# Autodesk Inventor assembly: Dash-V1
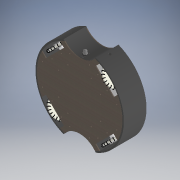
[picture p0: Inventor's stored thumbnail of the model, 180x180]
Saved by Autodesk Inventor 2020 (Build 240168000, 168)
## iProperties
Created: 2024-10-26
Part Number: Dash-V1
Document SubType Name: Assembly
Designer: Ivan
Mass: 1036.29 g
Surface Area: 3844.11 cm^2
Volume: 1024.75 cm^3
Density: 1.01126 g/cm^3
Author: Ivan
## Documents named in this file (13)
- C:\!projects\DASH_\3D\Dash-V1\Dash-V1.iam
- C:\!projects\DASH_\3D\Dash-V1\floor_v2.ipt
- C:\!projects\DASH_\3D\Dash-V1\motor_mount\motor_mount_edge_v2.ipt
- C:\!projects\DASH_\3D\Dash-V1\motor_mount\motor_converter.ipt
- C:\!projects\DASH_\3D\Dash-V1\motor_mount\motor_mount_part2_v2.ipt
- C:\!projects\DASH_\3D\Dash-V1\motor20.ipt
- C:\!projects\DASH_\3D\Dash-V1\wheel\Wheel.iam
- C:\!projects\DASH_\3D\Dash-V1\contour.ipt
- C:\!projects\DASH_\3D\Dash-V1\protect_v2.ipt
- C:\!projects\DASH_\3D\Dash-V1\ball.ipt
- C:\!projects\DASH_\3D\Dash-V1\catch_v2.ipt
- C:\!projects\DASH_\3D\Dash-V1\Solenoid\Solenoid.iam
- C:\!projects\DASH_\3D\Dash-V1\motherboard\motherboard_asm.iam
## Components (27 placed, 12 different names)
1. ball:1 — Касательность:1, Касательность:2
2. motherboard_asm:1 [sub-assembly] — Вставка:46, Вставка:47
3. floor_v2:1 — Совмещение:2, Вставка:1, Вставка:2, Совмещение:3, Угол:1, Вставка:3, Вставка:4, Вставка:10, Вставка:11, Вставка:12, Вставка:13, Вставка:14, Вставка:15, Вставка:16, Вставка:17, Вставка:18, Вставка:19, Вставка:20, Вставка:21, Касательность:1, Вставка:38, Вставка:39, Вставка:40, Вставка:41, Совмещение:4, Касательность:3, Касательность:4, Вставка:42, Вставка:43, Вставка:44, Вставка:45
4. contour:1 — Вставка:9, Касательность:2, Вставка:35, Вставка:46, Вставка:47
5. motor_converter:1 — Вставка:36, Вставка:37, Угол:3
6. motor_mount_edge_v2:2 — Вставка:18, Вставка:19, Вставка:24, Вставка:25, Вставка:28, Вставка:35
7. motor_mount_edge_v2:3 — Вставка:20, Вставка:21, Вставка:22, Вставка:23, Вставка:30
8. motor_mount_edge_v2:4 — Вставка:14, Вставка:15, Вставка:26, Вставка:27, Вставка:29
9. motor_mount_edge_v2:1 — Вставка:1, Вставка:2, Вставка:5, Вставка:6, Вставка:7, Вставка:9
10. motor_mount_part2_v2:5 — Вставка:16, Вставка:17
11. motor_mount_part2_v2:6 — Вставка:12, Вставка:13
12. motor_mount_part2_v2:7 — Вставка:10, Вставка:11, Вставка:37
13. motor_mount_part2_v2:4 — Вставка:3, Вставка:4, Вставка:36
14. motor20:2 — Вставка:22, Вставка:23
15. motor20:3 — Вставка:24, Вставка:25
16. motor20:4 — Вставка:26, Вставка:27
17. motor20:1 — Вставка:5, Вставка:6
18. Wheel:1 [sub-assembly] — Вставка:7
19. Wheel:2 [sub-assembly] — Вставка:30
20. Wheel:3 [sub-assembly] — Вставка:29
21. Wheel:4 [sub-assembly] — Вставка:28
22. catch_v2:2 — Вставка:40, Вставка:41
23. catch_v2:1 — Вставка:38, Вставка:39
24. protect_v2:2 — Вставка:44, Вставка:45
25. protect_v2:1 — Вставка:42, Вставка:43
26. Solenoid:2 [sub-assembly] — Угол:2, Заподлицо:1, Заподлицо:2, Касательность:4, Угол:3
27. Solenoid:1 [sub-assembly] — Угол:2, Заподлицо:1, Совмещение:4, Заподлицо:2, Касательность:3
## Relationships (54: Insert 42, Tangent 4, Mate 3, Angle 3, Flush 2)
- Совмещение:2 [Mate]: floor_v2:1
- Вставка:1 [Insert]: floor_v2:1 ↔ motor_mount_edge_v2:1
- Вставка:2 [Insert]: floor_v2:1 ↔ motor_mount_edge_v2:1
- Совмещение:3 [Mate]: floor_v2:1
- Угол:1 [Angle] (45 deg): floor_v2:1
- Вставка:3 [Insert]: floor_v2:1 ↔ motor_mount_part2_v2:4
- Вставка:4 [Insert]: floor_v2:1 ↔ motor_mount_part2_v2:4
- Вставка:5 [Insert]: motor_mount_edge_v2:1 ↔ motor20:1
- Вставка:6 [Insert]: motor_mount_edge_v2:1 ↔ motor20:1
- Вставка:7 [Insert]: motor_mount_edge_v2:1 ↔ Wheel:1
- Вставка:9 [Insert]: contour:1 ↔ motor_mount_edge_v2:1
- Вставка:10 [Insert]: floor_v2:1 ↔ motor_mount_part2_v2:7
- Вставка:11 [Insert]: floor_v2:1 ↔ motor_mount_part2_v2:7
- Вставка:12 [Insert]: floor_v2:1 ↔ motor_mount_part2_v2:6
- Вставка:13 [Insert]: floor_v2:1 ↔ motor_mount_part2_v2:6
- Вставка:14 [Insert]: floor_v2:1 ↔ motor_mount_edge_v2:4
- Вставка:15 [Insert]: floor_v2:1 ↔ motor_mount_edge_v2:4
- Вставка:16 [Insert]: floor_v2:1 ↔ motor_mount_part2_v2:5
- Вставка:17 [Insert]: floor_v2:1 ↔ motor_mount_part2_v2:5
- Вставка:18 [Insert]: floor_v2:1 ↔ motor_mount_edge_v2:2
- Вставка:19 [Insert]: floor_v2:1 ↔ motor_mount_edge_v2:2
- Вставка:20 [Insert]: floor_v2:1 ↔ motor_mount_edge_v2:3
- Вставка:21 [Insert]: floor_v2:1 ↔ motor_mount_edge_v2:3
- Вставка:22 [Insert]: motor_mount_edge_v2:3 ↔ motor20:2
- Вставка:23 [Insert]: motor_mount_edge_v2:3 ↔ motor20:2
- Вставка:24 [Insert]: motor_mount_edge_v2:2 ↔ motor20:3
- Вставка:25 [Insert]: motor_mount_edge_v2:2 ↔ motor20:3
- Вставка:26 [Insert]: motor_mount_edge_v2:4 ↔ motor20:4
- Вставка:27 [Insert]: motor_mount_edge_v2:4 ↔ motor20:4
- Вставка:28 [Insert]: motor_mount_edge_v2:2 ↔ Wheel:4
- Вставка:29 [Insert]: motor_mount_edge_v2:4 ↔ Wheel:3
- Вставка:30 [Insert]: motor_mount_edge_v2:3 ↔ Wheel:2
- Касательность:1 [Tangent]: ball:1 ↔ floor_v2:1
- Касательность:2 [Tangent]: ball:1 ↔ contour:1
- Вставка:35 [Insert]: contour:1 ↔ motor_mount_edge_v2:2
- Вставка:36 [Insert]: motor_converter:1 ↔ motor_mount_part2_v2:4
- Вставка:37 [Insert]: motor_converter:1 ↔ motor_mount_part2_v2:7
- Вставка:38 [Insert]: floor_v2:1 ↔ catch_v2:1
- Вставка:39 [Insert]: floor_v2:1 ↔ catch_v2:1
- Вставка:40 [Insert]: floor_v2:1 ↔ catch_v2:2
- Вставка:41 [Insert]: floor_v2:1 ↔ catch_v2:2
- Угол:2 [Angle] (180 deg): Solenoid:2 ↔ Solenoid:1
- Заподлицо:1 [Flush]: Solenoid:2 ↔ Solenoid:1
- Совмещение:4 [Mate]: floor_v2:1 ↔ Solenoid:1
- Заподлицо:2 [Flush]: Solenoid:2 ↔ Solenoid:1
- Касательность:3 [Tangent]: floor_v2:1 ↔ Solenoid:1
- Касательность:4 [Tangent]: floor_v2:1 ↔ Solenoid:2
- Угол:3 [Angle] (0 deg): motor_converter:1 ↔ Solenoid:2
- Вставка:42 [Insert]: floor_v2:1 ↔ protect_v2:1
- Вставка:43 [Insert]: floor_v2:1 ↔ protect_v2:1
- Вставка:44 [Insert]: floor_v2:1 ↔ protect_v2:2
- Вставка:45 [Insert]: floor_v2:1 ↔ protect_v2:2
- Вставка:46 [Insert]: motherboard_asm:1 ↔ contour:1
- Вставка:47 [Insert]: motherboard_asm:1 ↔ contour:1
